# Autodesk Inventor assembly: Caja actor-re-actor engranes acrílicos
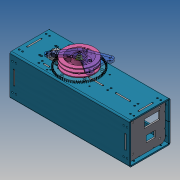
[picture p0: Inventor's stored thumbnail of the model, 180x180]
Saved by Autodesk Inventor 2017 (Build 210142000, 142)
## iProperties
Part Number: Caja actor-re-actor engranes acrílicos
Material: Genérico
Document SubType Name: Assembly
Designer: Leo
Author: Leo
## Documents named in this file (6)
- C:\Users\Leo\Dropbox\E\Caja Motriz\Caja actor-re-actor engranes acrílicos.iam
- C:\Users\Leo\Dropbox\E\Caja Motriz\Piezas\Motor.ipt
- C:\Users\Leo\Dropbox\E\Caja Motriz\transmision Engranajes\Design Accelerator\Engranajes rectos1.iam
- C:\Users\Leo\Dropbox\E\Caja Motriz\transmision Engranajes\Conjunto Polea.iam
- C:\Users\Leo\Dropbox\E\Caja Motriz\CaseB.iam
- C:\Users\Leo\Dropbox\E\Caja Motriz\transmision Engranajes\Plato Carrete-doble.iam
## Components (5 placed, 5 different names)
1. CaseB:1 [sub-assembly] — Nivelación:10, Nivelación:2, Nivelación:3, Coincidencia:1, Coincidencia:10
2. Motor:1 — Nivelación:4, Nivelación:5, Nivelación:6, Insertar:1
3. Plato Carrete-doble:1 [sub-assembly] — Coincidencia:1, Coincidencia:10
4. Conjunto Polea:1 [sub-assembly] — Insertar:1
5. Engranajes rectos:1 [sub-assembly]
## Relationships (9: Flush 6, Mate 2, Insert 1)
- Nivelación:10 [Flush]: CaseB:1
- Nivelación:2 [Flush]: CaseB:1
- Nivelación:3 [Flush]: CaseB:1
- Nivelación:4 [Flush]: Motor:1
- Nivelación:5 [Flush]: Motor:1
- Nivelación:6 [Flush] (5 mm): Motor:1
- Insertar:1: Motor:1 ↔ Conjunto Polea:1
- Coincidencia:1 [Mate]: CaseB:1 ↔ Plato Carrete-doble:1
- Coincidencia:10 [Mate] (2 mm): CaseB:1 ↔ Plato Carrete-doble:1
